# Autodesk Inventor assembly: Nanoscopy-on-a-cheap_v3_mono
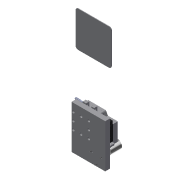
[picture p0: Inventor's stored thumbnail of the model, 180x180]
Saved by Autodesk Inventor 2019 (Build 230136000, 136)
## iProperties
Created: 2019-05-02
Part Number: Nanoscopy-on-a-cheap_v3_mono
Document SubType Name: Assembly
Designer: diederichbenedict
Author: diederichbenedict
## Documents named in this file (12)
- C:\Users\diederichbenedict\Dropbox\Dokumente\Promotion\PROJECTS\STORMoChip\INVENTOR\Nanoscopy-on-a-cheap\Nanoscopy-on-a-cheap_v3_mono.iam
- C:\Users\diederichbenedict\Dropbox\Dokumente\Promotion\PROJECTS\STORMoChip\INVENTOR\Nanoscopy-on-a-cheap\00_ZEISS_Axiotech_Plate.ipt
- C:\Users\diederichbenedict\Dropbox\Dokumente\Promotion\PROJECTS\STORMoChip\INVENTOR\Nanoscopy-on-a-cheap\00_XY_stage-CHUO_SEIKI_LD-647-R1.iam
- C:\Users\diederichbenedict\Dropbox\Dokumente\Promotion\PROJECTS\STORMoChip\INVENTOR\Nanoscopy-on-a-cheap\Assembly_Lasergroup_wPickup_v1.iam
- C:\Users\diederichbenedict\Dropbox\Dokumente\Promotion\PROJECTS\STORMoChip\INVENTOR\Nanoscopy-on-a-cheap\00_Microscope_Objective.ipt
- C:\Users\diederichbenedict\Dropbox\Dokumente\Promotion\PROJECTS\STORMoChip\INVENTOR\Nanoscopy-on-a-cheap\10_Adapter_Laser_XY_left.ipt
- C:\Users\diederichbenedict\Dropbox\Dokumente\Promotion\PROJECTS\STORMoChip\INVENTOR\Nanoscopy-on-a-cheap\02_Nanoscopy_Chip.ipt
- C:\Users\diederichbenedict\Dropbox\Dokumente\Promotion\PROJECTS\STORMoChip\INVENTOR\Nanoscopy-on-a-cheap\10_Baseplate.ipt
- C:\Users\diederichbenedict\Dropbox\Dokumente\Promotion\PROJECTS\STORMoChip\INVENTOR\Nanoscopy-on-a-cheap\00_Baseplate_Axiotech.ipt
- C:\Users\diederichbenedict\Dropbox\Dokumente\Promotion\PROJECTS\STORMoChip\INVENTOR\Nanoscopy-on-a-cheap\10_Baseplate_Axiotech_mono.ipt
- C:\Users\diederichbenedict\Documents\Inventor\Content Center Files\R2019\en-US\DIN 912\DIN 912 - M3 x 0.5 x 20 x 18.75.ipt
- C:\Users\diederichbenedict\Dropbox\Dokumente\Promotion\PROJECTS\STORMoChip\INVENTOR\Nanoscopy-on-a-cheap\00_Ballmagnets_5mm.ipt
## Components (13 placed, 11 different names)
1. 00_ZEISS_Axiotech_Plate:1 — Mate:13
2. 00_XY_stage-CHUO_SEIKI_LD-647-R1:1 [sub-assembly] — Flush:6, Flush:11, Flush:12, Flush:22, Flush:23, Flush:24, Flush:25, Flush:26
3. Assembly_Lasergroup_wPickup_v1:2 [sub-assembly] — Flush:6, Mate:7, Mate:8
4. 02_Nanoscopy_Chip:1
5. 00_Microscope_Objective:1 — Mate:7, Mate:8, Mate:13
6. 10_Adapter_Laser_XY_left:1 — Flush:11, Flush:12
7. 10_Baseplate:1 — Flush:22, Flush:23
8. 00_Baseplate_Axiotech:1
9. 10_Baseplate_Axiotech_mono:1 — Flush:24, Flush:25, Flush:26, Mate:15, Mate:16
10. DIN 912 - replaced by DIN EN ISO 4762 M3 x 20:1 — Mate:14, Mate:16
11. DIN 912 - replaced by DIN EN ISO 4762 M3 x 20:2 — Mate:15
12. DIN 912 - replaced by DIN EN ISO 4762 M3 x 20:3
13. 00_Ballmagnets_5mm:1 — Mate:14
## Relationships (16: Flush 8, Mate 6, Insert 1, Angle 1)
- Flush:6: 00_XY_stage-CHUO_SEIKI_LD-647-R1:1 ↔ Assembly_Lasergroup_wPickup_v1:2
- Mate:7 (30 mm): Assembly_Lasergroup_wPickup_v1:2 ↔ 00_Microscope_Objective:1
- Mate:8 (-16 mm): Assembly_Lasergroup_wPickup_v1:2 ↔ 00_Microscope_Objective:1
- Flush:11: 00_XY_stage-CHUO_SEIKI_LD-647-R1:1 ↔ 10_Adapter_Laser_XY_left:1
- Flush:12: 00_XY_stage-CHUO_SEIKI_LD-647-R1:1 ↔ 10_Adapter_Laser_XY_left:1
- Mate:13 (30 mm): 00_ZEISS_Axiotech_Plate:1 ↔ 00_Microscope_Objective:1
- [Insert] (5 mm): 02_Nanoscopy_Chip:1 ↔ 00_Microscope_Objective:1
- [Angle] (180 deg): 02_Nanoscopy_Chip:1 ↔ 10_Adapter_Laser_XY_left:1
- Flush:22: 00_XY_stage-CHUO_SEIKI_LD-647-R1:1 ↔ 10_Baseplate:1
- Flush:23: 00_XY_stage-CHUO_SEIKI_LD-647-R1:1 ↔ 10_Baseplate:1
- Flush:24: 00_XY_stage-CHUO_SEIKI_LD-647-R1:1 ↔ 10_Baseplate_Axiotech_mono:1
- Flush:25: 00_XY_stage-CHUO_SEIKI_LD-647-R1:1 ↔ 10_Baseplate_Axiotech_mono:1
- Flush:26: 00_XY_stage-CHUO_SEIKI_LD-647-R1:1 ↔ 10_Baseplate_Axiotech_mono:1
- Mate:14: DIN 912 - replaced by DIN EN ISO 4762 M3 x 20:1 ↔ 00_Ballmagnets_5mm:1
- Mate:15: 10_Baseplate_Axiotech_mono:1 ↔ DIN 912 - replaced by DIN EN ISO 4762 M3 x 20:2
- Mate:16: 10_Baseplate_Axiotech_mono:1 ↔ DIN 912 - replaced by DIN EN ISO 4762 M3 x 20:1
